# Autodesk Inventor assembly: Pedal Assembly
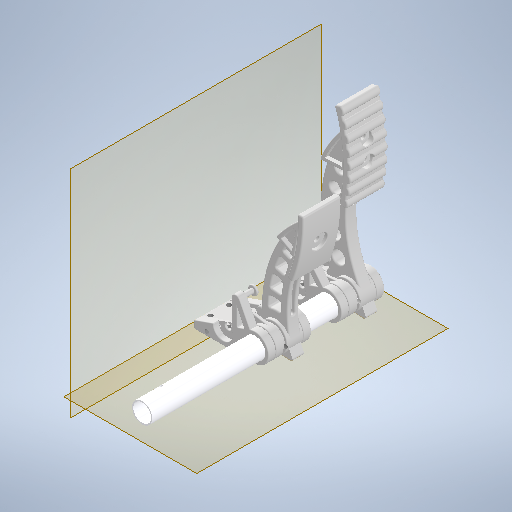
[picture p0: Inventor's stored thumbnail of the model, 512x512]
Saved by Autodesk Inventor 2025.2 (Build 292293000, 293)
## iProperties
Created: 2025-03-25
Part Number: Pedal Assembly
Document SubType Name: Assembly
Designer: eason
Author: eason
## Documents named in this file (10)
- C:\Users\eason\Desktop\Code\Unojoy-Simulator-Rig\CAD\Pedals\Pedal Assembly.iam
- C:\Users\eason\Desktop\Code\Unojoy-Simulator-Rig\CAD\Pedals\Pedal Arm.ipt
- C:\Users\eason\Desktop\Code\Unojoy-Simulator-Rig\CAD\Pedals\Pedal Face.ipt
- C:\Users\eason\Desktop\Code\Unojoy-Simulator-Rig\CAD\Pedals\Pedal Support Base.ipt
- C:\Users\eason\Desktop\Code\Unojoy-Simulator-Rig\CAD\Pedals\Pedal Support L.ipt
- C:\Users\eason\Desktop\Code\Unojoy-Simulator-Rig\CAD\Pedals\Pedal Support R.ipt
- C:\Users\eason\Desktop\Code\Unojoy-Simulator-Rig\CAD\Pedals\Steering PVC.ipt
- C:\Users\eason\Desktop\Code\Unojoy-Simulator-Rig\CAD\Pedals\Pedal Arm Short.ipt
- C:\Users\eason\Desktop\Code\Unojoy-Simulator-Rig\CAD\Pedals\Pedal Face Short.ipt
- C:\Users\eason\Desktop\Code\Unojoy-Simulator-Rig\CAD\Pedals\Pedal Support L New.ipt
## Components (11 placed, 9 different names)
1. Pedal Arm:1 — Cylindrical:3, Mate:8, Cylindrical:4, Cylindrical:5, Mate:9, Angle:2
2. Pedal Face:1 — Cylindrical:4, Cylindrical:5, Mate:9
3. Pedal Support Base:1 — Mate:1, Mate:2, Mate:3, Mate:6, Mate:7, Cylindrical:1, Cylindrical:2
4. Pedal Support L:1 — Mate:4, Mate:6, Cylindrical:1, Mate:12
5. Pedal Support R:1 — Mate:5, Mate:7, Cylindrical:2, Insert:1, Mate:8
6. Steering PVC:1 — Insert:1, Cylindrical:3, Cylindrical:8
7. Pedal Arm Short:1 — Mate:17, Cylindrical:8, Cylindrical:9, Angle:1, Mate:18, Angle:2
8. Pedal Face Short:1 — Cylindrical:9, Angle:1, Mate:18
9. Pedal Support L New:1 — Mate:14, Mate:16, Cylindrical:6
10. Pedal Support Base:2 — Mate:10, Mate:11, Mate:12, Mate:15, Mate:16, Cylindrical:6, Cylindrical:7
11. Pedal Support R:2 — Mate:13, Mate:15, Cylindrical:7, Mate:17
## Relationships (30: Mate 18, CylindricalJoint 9, Angle 2, Insert 1)
- Mate:1: Pedal Support Base:1
- Mate:2: Pedal Support Base:1
- Mate:3: Pedal Support Base:1
- Mate:4: Pedal Support L:1
- Mate:5: Pedal Support R:1
- Mate:6: Pedal Support Base:1 ↔ Pedal Support L:1
- Mate:7: Pedal Support Base:1 ↔ Pedal Support R:1
- Cylindrical:1: Pedal Support Base:1 ↔ Pedal Support L:1
- Cylindrical:2: Pedal Support Base:1 ↔ Pedal Support R:1
- Insert:1: Pedal Support R:1 ↔ Steering PVC:1
- Cylindrical:3: Pedal Arm:1 ↔ Steering PVC:1
- Mate:8 (0.02 mm): Pedal Arm:1 ↔ Pedal Support R:1
- Cylindrical:4: Pedal Arm:1 ↔ Pedal Face:1
- Cylindrical:5: Pedal Arm:1 ↔ Pedal Face:1
- Mate:9: Pedal Arm:1 ↔ Pedal Face:1
- Mate:10: Pedal Support Base:2
- Mate:11: Pedal Support Base:2
- Mate:12 (50 mm): Pedal Support L:1 ↔ Pedal Support Base:2
- Mate:13: Pedal Support R:2
- Mate:14: Pedal Support L New:1
- Mate:15: Pedal Support Base:2 ↔ Pedal Support R:2
- Mate:16: Pedal Support L New:1 ↔ Pedal Support Base:2
- Cylindrical:6: Pedal Support L New:1 ↔ Pedal Support Base:2
- Cylindrical:7: Pedal Support Base:2 ↔ Pedal Support R:2
- Mate:17 (0.02 mm): Pedal Arm Short:1 ↔ Pedal Support R:2
- Cylindrical:8: Steering PVC:1 ↔ Pedal Arm Short:1
- Cylindrical:9: Pedal Arm Short:1 ↔ Pedal Face Short:1
- Angle:1 (0 deg): Pedal Arm Short:1 ↔ Pedal Face Short:1
- Mate:18: Pedal Arm Short:1 ↔ Pedal Face Short:1
- Angle:2 (0 deg): Pedal Arm:1 ↔ Pedal Arm Short:1
